# Autodesk Inventor assembly: Assembly_Spiral_XY_MGN7
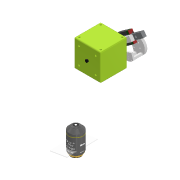
[picture p0: Inventor's stored thumbnail of the model, 180x180]
Saved by Autodesk Inventor 2022 (Build 260153000, 153)
## iProperties
Created: 2023-09-18
Part Number: Assembly_Spiral_XY_MGN7
Document SubType Name: Assembly
Designer: diederichbenedict
Author: diederichbenedict
## Documents named in this file (12)
- C:\Users\diederichbenedict\Dropbox\Dokumente\Promotion\PROJECTS\openUC2-CAD\INVENTOR\Assembly_Spiral_XY_MGN7.iam
- Assembly_Spiral_XY_MGN9.iam
- C:\Users\diederichbenedict\Dropbox\Dokumente\Promotion\PROJECTS\openUC2-CAD\INVENTOR\55_spiralxy_spiral.ipt
- C:\Users\diederichbenedict\Dropbox\Dokumente\Promotion\PROJECTS\openUC2-CAD\INVENTOR\00_Sample_Doubleslit.ipt
- C:\Users\diederichbenedict\Dropbox\Dokumente\Promotion\PROJECTS\openUC2-CAD\INVENTOR\00_Microscope_objective_4x.ipt
- C:\Users\diederichbenedict\Dropbox\Dokumente\Promotion\PROJECTS\openUC2-CAD\INVENTOR\00_NEMA_17.ipt
- C:\Users\diederichbenedict\Dropbox\Dokumente\Promotion\PROJECTS\openUC2-CAD\INVENTOR\00_Actuator_MGN9C.ipt
- C:\Users\diederichbenedict\Dropbox\Dokumente\Promotion\PROJECTS\openUC2-CAD\INVENTOR\00_Actuator_MGN9.ipt
- C:\Users\diederichbenedict\Dropbox\Dokumente\Promotion\PROJECTS\openUC2-CAD\INVENTOR\55_spiralxy_motormount_NEMA_MGN7.ipt
- C:\Users\diederichbenedict\Dropbox\Dokumente\Promotion\PROJECTS\openUC2-CAD\INVENTOR\55_spiralxy_motorplate_nema_mgn9.ipt
- C:\Users\diederichbenedict\Dropbox\Dokumente\Promotion\PROJECTS\openUC2-CAD\INVENTOR\tmp_rotatingstage\55_spiralxy_slidemount_MGN7.ipt
- C:\Users\diederichbenedict\Dropbox\Dokumente\Promotion\PROJECTS\openUC2-CAD\INVENTOR\55_spiralxy_slidemount_MGN9_Nema17_Body.ipt
## Components (11 placed, 10 different names)
1. 55_spiralxy_motormount_NEMA_MGN7:1 — Passend:8, Passend:9, Passend:10, Einfügen:9
2. 00_Sample_Doubleslit:1
3. 00_Microscope_objective_4x:1
4. 00_NEMA_17:1
5. 00_Actuator_MGN9C:1 — Passend:6, Passend:7, Passend:11, Einfügen:10
6. 00_Actuator_MGN9:1 — Passend:6, Passend:7, Passend:8, Passend:9, Passend:10, Passend:11
7. 55_spiralxy_slidemount_MGN7:1 — Einfügen:10
8. 55_spiralxy_slidemount_MGN9_Nema17_Body:1 — Passend:12, Winkel:3, Passend:13
9. 00_NEMA_17:2 — Passend:12, Winkel:3, Passend:13, Einfügen:7, Winkel:4, Winkel:5, Einfügen:9
10. 55_spiralxy_motorplate_nema_mgn9:1 — Einfügen:7, Winkel:4, Einfügen:8
11. 55_spiralxy_spiral:1 — Einfügen:8, Winkel:5
## Relationships (15: Mate 8, Insert 4, Angle 3)
- Passend:6 [Mate]: 00_Actuator_MGN9C:1 ↔ 00_Actuator_MGN9:1
- Passend:7 [Mate]: 00_Actuator_MGN9C:1 ↔ 00_Actuator_MGN9:1
- Passend:8 [Mate]: 55_spiralxy_motormount_NEMA_MGN7:1 ↔ 00_Actuator_MGN9:1
- Passend:9 [Mate]: 55_spiralxy_motormount_NEMA_MGN7:1 ↔ 00_Actuator_MGN9:1
- Passend:10 [Mate]: 55_spiralxy_motormount_NEMA_MGN7:1 ↔ 00_Actuator_MGN9:1
- Passend:11 [Mate]: 00_Actuator_MGN9C:1 ↔ 00_Actuator_MGN9:1
- Passend:12 [Mate]: 55_spiralxy_slidemount_MGN9_Nema17_Body:1 ↔ 00_NEMA_17:2
- Winkel:3 [Angle] (180 deg): 55_spiralxy_slidemount_MGN9_Nema17_Body:1 ↔ 00_NEMA_17:2
- Passend:13 [Mate]: 55_spiralxy_slidemount_MGN9_Nema17_Body:1 ↔ 00_NEMA_17:2
- Einfügen:7 [Insert]: 00_NEMA_17:2 ↔ 55_spiralxy_motorplate_nema_mgn9:1
- Winkel:4 [Angle] (180 deg): 00_NEMA_17:2 ↔ 55_spiralxy_motorplate_nema_mgn9:1
- Einfügen:8 [Insert]: 55_spiralxy_motorplate_nema_mgn9:1 ↔ 55_spiralxy_spiral:1
- Winkel:5 [Angle] (0 deg): 00_NEMA_17:2 ↔ 55_spiralxy_spiral:1
- Einfügen:9 [Insert]: 55_spiralxy_motormount_NEMA_MGN7:1 ↔ 00_NEMA_17:2
- Einfügen:10 [Insert]: 00_Actuator_MGN9C:1 ↔ 55_spiralxy_slidemount_MGN7:1
